# Autodesk Inventor assembly: Lidar Sensor Lexan Assembly
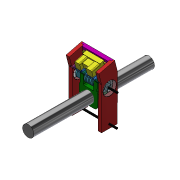
[picture p0: Inventor's stored thumbnail of the model, 180x180]
Saved by Autodesk Inventor 2018.3 (Build 223284000, 284)
## iProperties
Created: 2019-02-26
Part Number: Lidar Sensor Lexan Assembly
Document SubType Name: Assembly
Designer: aye06091
Mass: 114.901 g
Surface Area: 461.678 cm^2
Volume: 114.901 cm^3
Density: 1 g/cm^3
Author: aye06091
## Documents named in this file (11)
- Y:\DeSimony-R\Senior R&D\4 R&D Shared Folder\VisiStick\VisiStick (Inventor)\Case Final\Lidar Sensor Lexan Assembly.iam
- Y:\DeSimony-R\Senior R&D\4 R&D Shared Folder\VisiStick\VisiStick (Inventor)\Case Final\Lidar Sensor CAse Piece 1.ipt
- Y:\DeSimony-R\Senior R&D\4 R&D Shared Folder\VisiStick\VisiStick (Inventor)\Case Final\Lidar Sensor Case Piece 2.ipt
- Y:\DeSimony-R\Senior R&D\4 R&D Shared Folder\VisiStick\VisiStick (Inventor)\Case Final\Lidar Sensor Case Piece 3.ipt
- Y:\DeSimony-R\Senior R&D\4 R&D Shared Folder\VisiStick\VisiStick (Inventor)\Electronics\Sharp 2Y0A02.ipt
- Y:\DeSimony-R\Senior R&D\4 R&D Shared Folder\VisiStick\VisiStick (Inventor)\Physical Parts\Lidar Sensor Case 4 v2.ipt
- Y:\DeSimony-R\Senior R&D\4 R&D Shared Folder\VisiStick\VisiStick (Inventor)\Case Final\Ball Bearing.ipt
- Y:\DeSimony-R\Senior R&D\4 R&D Shared Folder\VisiStick\VisiStick (Inventor)\Case Final\Steel Rod.ipt
- Y:\DeSimony-R\Senior R&D\4 R&D Shared Folder\VisiStick\VisiStick (Inventor)\Physical Parts\T-Spacer .125 inch bore.ipt
- Y:\DeSimony-R\Senior R&D\4 R&D Shared Folder\VisiStick\VisiStick (Inventor)\Physical Parts\Cane Segmant.ipt
- \\niskyschools.org\dfs\Student\Home\GY2019\aye06091\Desktop\Copy of Sensor Model\Smaller Needle Bearing Mount.ipt
## Components (17 placed, 10 different names)
1. Sharp 2Y0A02:1 — Insert:5, Insert:6
2. Lidar Sensor CAse Piece 1:1 — Insert:24, Flush:4, Mate:16, Mate:17, Flush:5, Mate:19, Insert:25
3. Lidar Sensor Case Piece 2:1 — Insert:9, Mate:12, Flush:3, Mate:18, Flush:6
4. Ball Bearing:1 — Insert:9, Insert:18
5. Ball Bearing:2 — Insert:11, Insert:19, Insert:25
6. Steel Rod:1 — Insert:11, Mate:6, Mate:13
7. Lidar Sensor Case 4 v2:1 — Mate:16, Mate:17, Flush:5, Mate:18, Flush:6
8. Lidar Sensor Case Piece 3:1 — Insert:5, Insert:6, Mate:12, Flush:3, Flush:4, Mate:19
9. T-Spacer .125 inch bore:1 — Insert:16
10. T-Spacer .125 inch bore:2 — Insert:18
11. T-Spacer .125 inch bore:3 — Insert:19
12. T-Spacer .125 inch bore:4 — Insert:16, Insert:17
13. T-Spacer .125 inch bore:5 — Insert:17, Insert:23
14. Cane Segmant:1 — Insert:21
15. Smaller Needle Bearing Mount:1 — Mate:6, Mate:13, Insert:21, Insert:22
16. T-Spacer .125 inch bore:6 — Insert:22, Insert:23
17. Steel Rod:2 — Insert:24
## Relationships (24: Insert 13, Mate 7, Flush 4)
- Insert:5: Sharp 2Y0A02:1 ↔ Lidar Sensor Case Piece 3:1
- Insert:6: Sharp 2Y0A02:1 ↔ Lidar Sensor Case Piece 3:1
- Insert:9: Lidar Sensor Case Piece 2:1 ↔ Ball Bearing:1
- Insert:11 (12.7 mm): Ball Bearing:2 ↔ Steel Rod:1
- Insert:16: T-Spacer .125 inch bore:1 ↔ T-Spacer .125 inch bore:4
- Insert:17: T-Spacer .125 inch bore:4 ↔ T-Spacer .125 inch bore:5
- Mate:6: Steel Rod:1 ↔ Smaller Needle Bearing Mount:1
- Insert:18: Ball Bearing:1 ↔ T-Spacer .125 inch bore:2
- Insert:19: Ball Bearing:2 ↔ T-Spacer .125 inch bore:3
- Mate:12: Lidar Sensor Case Piece 2:1 ↔ Lidar Sensor Case Piece 3:1
- Flush:3: Lidar Sensor Case Piece 2:1 ↔ Lidar Sensor Case Piece 3:1
- Mate:13: Steel Rod:1 ↔ Smaller Needle Bearing Mount:1
- Insert:21 (-101.6 mm): Cane Segmant:1 ↔ Smaller Needle Bearing Mount:1
- Insert:22: Smaller Needle Bearing Mount:1 ↔ T-Spacer .125 inch bore:6
- Insert:23: T-Spacer .125 inch bore:5 ↔ T-Spacer .125 inch bore:6
- Insert:24 (-12.7 mm): Lidar Sensor CAse Piece 1:1 ↔ Steel Rod:2
- Flush:4: Lidar Sensor CAse Piece 1:1 ↔ Lidar Sensor Case Piece 3:1
- Mate:16: Lidar Sensor CAse Piece 1:1 ↔ Lidar Sensor Case 4 v2:1
- Mate:17: Lidar Sensor CAse Piece 1:1 ↔ Lidar Sensor Case 4 v2:1
- Flush:5: Lidar Sensor CAse Piece 1:1 ↔ Lidar Sensor Case 4 v2:1
- Mate:18: Lidar Sensor Case Piece 2:1 ↔ Lidar Sensor Case 4 v2:1
- Flush:6: Lidar Sensor Case Piece 2:1 ↔ Lidar Sensor Case 4 v2:1
- Mate:19: Lidar Sensor CAse Piece 1:1 ↔ Lidar Sensor Case Piece 3:1
- Insert:25: Lidar Sensor CAse Piece 1:1 ↔ Ball Bearing:2
